# Autodesk Inventor assembly: 조립품2
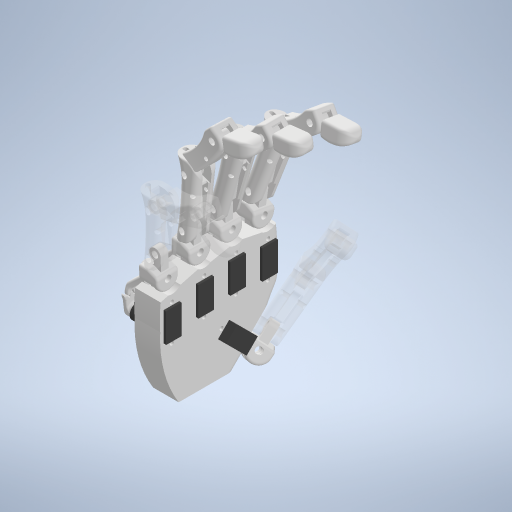
[picture p0: Inventor's stored thumbnail of the model, 512x512]
Saved by Autodesk Inventor 2024 (Build 280153000, 153)
## iProperties
Created: 2023-05-16
Part Number: 조립품2
Document SubType Name: Assembly
Designer: Lenovo
Author: Lenovo
## Documents named in this file (12)
- C:\Users\Lenovo\OneDrive\바탕 화면\로봇손\조립품2.iam
- C:\Users\Lenovo\OneDrive\바탕 화면\로봇손\손바닥.ipt
- C:\Users\Lenovo\OneDrive\바탕 화면\로봇손\손바닥 모터.ipt
- C:\Users\Lenovo\OneDrive\바탕 화면\로봇손\2,4 아래.ipt
- C:\Users\Lenovo\OneDrive\바탕 화면\로봇손\손바닥 위 -2.ipt
- C:\Users\Lenovo\OneDrive\바탕 화면\로봇손\3 아래.ipt
- C:\Users\Lenovo\OneDrive\바탕 화면\로봇손\중간.ipt
- C:\Users\Lenovo\OneDrive\바탕 화면\로봇손\위.ipt
- C:\Users\Lenovo\OneDrive\바탕 화면\로봇손\손바닥 위.ipt
- C:\Users\Lenovo\OneDrive\바탕 화면\로봇손\5 아래.ipt
- C:\Users\Lenovo\OneDrive\바탕 화면\로봇손\엄지 기어 -2.ipt
- C:\Users\Lenovo\OneDrive\바탕 화면\로봇손\손가락 기어.ipt
## Components (31 placed, 11 different names)
1. 손바닥:1 — 메이트:17, 메이트:18, 메이트:24, 메이트:27, 메이트:30, 메이트:36, 메이트:51, 메이트:52, 메이트:53, 메이트:54, 메이트:83, 메이트:84, 메이트:85, 메이트:86, 메이트:87, 메이트:88, 메이트:91, 메이트:92, 메이트:93, 메이트:96, 메이트:97, 메이트:98, 메이트:99, 메이트:100, 메이트:101
2. 손바닥 모터:4 — 메이트:17, 메이트:18, 메이트:36, 메이트:103, 메이트:107
3. 손바닥 모터:5 — 메이트:24, 메이트:27, 메이트:30, 메이트:102, 메이트:106
4. 손바닥 위 -2:4 — 메이트:79, 메이트:80, 메이트:83, 메이트:84
5. 중간:1 — 메이트:49, 메이트:50, 메이트:81, 메이트:82
6. 위:1 — 메이트:49, 메이트:50
7. 손바닥 위:1 — 메이트:51, 메이트:53, 메이트:57, 메이트:59
8. 손바닥 위:2 — 메이트:52, 메이트:54, 메이트:55, 메이트:56
9. 2,4 아래:2 — 메이트:57, 메이트:59, 메이트:65, 메이트:69
10. 2,4 아래:3 — 메이트:63, 메이트:67, 메이트:89
11. 5 아래:1 — 메이트:55, 메이트:56, 메이트:66, 메이트:70
12. 3 아래:2 — 메이트:64, 메이트:68, 메이트:90
13. 중간:2 — 메이트:63, 메이트:67, 메이트:71, 메이트:75
14. 중간:3 — 메이트:64, 메이트:68, 메이트:72, 메이트:76
15. 중간:4 — 메이트:65, 메이트:69, 메이트:73, 메이트:77
16. 중간:5 — 메이트:66, 메이트:70, 메이트:74, 메이트:78
17. 위:2 — 메이트:74, 메이트:78
18. 위:3 — 메이트:73, 메이트:77
19. 위:4 — 메이트:72, 메이트:76
20. 위:5 — 메이트:71, 메이트:75
21. 5 아래:2 — 메이트:79, 메이트:80, 메이트:81, 메이트:82
22. 손바닥 위:3 — 메이트:86, 메이트:87, 메이트:89
23. 손바닥 위:4 — 메이트:85, 메이트:88, 메이트:90
24. 손바닥 모터:9 — 메이트:91, 메이트:92, 메이트:93, 메이트:94, 메이트:95
25. 엄지 기어 -2:1 — 메이트:94, 메이트:95
26. 손바닥 모터:10 — 메이트:96, 메이트:97, 메이트:101, 메이트:104, 메이트:108
27. 손바닥 모터:11 — 메이트:98, 메이트:99, 메이트:100, 메이트:105, 메이트:109
28. 손가락 기어:1 — 메이트:102, 메이트:106
29. 손가락 기어:2 — 메이트:103, 메이트:107
30. 손가락 기어:3 — 메이트:104, 메이트:108
31. 손가락 기어:4 — 메이트:105, 메이트:109
## Relationships (63: Mate 63)
- 메이트:17 [Mate]: 손바닥:1 ↔ 손바닥 모터:4
- 메이트:18 [Mate]: 손바닥:1 ↔ 손바닥 모터:4
- 메이트:24 [Mate]: 손바닥:1 ↔ 손바닥 모터:5
- 메이트:27 [Mate]: 손바닥:1 ↔ 손바닥 모터:5
- 메이트:30 [Mate]: 손바닥:1 ↔ 손바닥 모터:5
- 메이트:36 [Mate]: 손바닥:1 ↔ 손바닥 모터:4
- 메이트:49 [Mate]: 중간:1 ↔ 위:1
- 메이트:50 [Mate] (0.5 mm): 중간:1 ↔ 위:1
- 메이트:51 [Mate]: 손바닥:1 ↔ 손바닥 위:1
- 메이트:52 [Mate]: 손바닥:1 ↔ 손바닥 위:2
- 메이트:53 [Mate] (0.5 mm): 손바닥:1 ↔ 손바닥 위:1
- 메이트:54 [Mate] (0.5 mm): 손바닥:1 ↔ 손바닥 위:2
- 메이트:55 [Mate]: 손바닥 위:2 ↔ 5 아래:1
- 메이트:56 [Mate] (0.5 mm): 손바닥 위:2 ↔ 5 아래:1
- 메이트:57 [Mate]: 손바닥 위:1 ↔ 2,4 아래:2
- 메이트:59 [Mate] (0.5 mm): 손바닥 위:1 ↔ 2,4 아래:2
- 메이트:63 [Mate]: 2,4 아래:3 ↔ 중간:2
- 메이트:64 [Mate]: 3 아래:2 ↔ 중간:3
- 메이트:65 [Mate]: 2,4 아래:2 ↔ 중간:4
- 메이트:66 [Mate]: 5 아래:1 ↔ 중간:5
- 메이트:67 [Mate] (0.5 mm): 2,4 아래:3 ↔ 중간:2
- 메이트:68 [Mate] (0.5 mm): 3 아래:2 ↔ 중간:3
- 메이트:69 [Mate] (0.5 mm): 2,4 아래:2 ↔ 중간:4
- 메이트:70 [Mate] (0.5 mm): 5 아래:1 ↔ 중간:5
- 메이트:71 [Mate]: 중간:2 ↔ 위:5
- 메이트:72 [Mate]: 중간:3 ↔ 위:4
- 메이트:73 [Mate]: 중간:4 ↔ 위:3
- 메이트:74 [Mate]: 중간:5 ↔ 위:2
- 메이트:75 [Mate] (0.5 mm): 중간:2 ↔ 위:5
- 메이트:76 [Mate] (0.5 mm): 중간:3 ↔ 위:4
- 메이트:77 [Mate] (0.5 mm): 중간:4 ↔ 위:3
- 메이트:78 [Mate] (0.5 mm): 중간:5 ↔ 위:2
- 메이트:79 [Mate]: 손바닥 위 -2:4 ↔ 5 아래:2
- 메이트:80 [Mate] (0.5 mm): 손바닥 위 -2:4 ↔ 5 아래:2
- 메이트:81 [Mate]: 중간:1 ↔ 5 아래:2
- 메이트:82 [Mate] (0.5 mm): 중간:1 ↔ 5 아래:2
- 메이트:83 [Mate]: 손바닥:1 ↔ 손바닥 위 -2:4
- 메이트:84 [Mate] (0.5 mm): 손바닥:1 ↔ 손바닥 위 -2:4
- 메이트:85 [Mate]: 손바닥:1 ↔ 손바닥 위:4
- 메이트:86 [Mate]: 손바닥:1 ↔ 손바닥 위:3
- 메이트:87 [Mate] (0.5 mm): 손바닥:1 ↔ 손바닥 위:3
- 메이트:88 [Mate] (0.5 mm): 손바닥:1 ↔ 손바닥 위:4
- 메이트:89 [Mate]: 2,4 아래:3 ↔ 손바닥 위:3
- 메이트:90 [Mate]: 3 아래:2 ↔ 손바닥 위:4
- 메이트:91 [Mate]: 손바닥:1 ↔ 손바닥 모터:9
- 메이트:92 [Mate]: 손바닥:1 ↔ 손바닥 모터:9
- 메이트:93 [Mate]: 손바닥:1 ↔ 손바닥 모터:9
- 메이트:94 [Mate]: 손바닥 모터:9 ↔ 엄지 기어 -2:1
- 메이트:95 [Mate] (0.5 mm): 손바닥 모터:9 ↔ 엄지 기어 -2:1
- 메이트:96 [Mate]: 손바닥:1 ↔ 손바닥 모터:10
- 메이트:97 [Mate]: 손바닥:1 ↔ 손바닥 모터:10
- 메이트:98 [Mate]: 손바닥:1 ↔ 손바닥 모터:11
- 메이트:99 [Mate]: 손바닥:1 ↔ 손바닥 모터:11
- 메이트:100 [Mate]: 손바닥:1 ↔ 손바닥 모터:11
- 메이트:101 [Mate]: 손바닥:1 ↔ 손바닥 모터:10
- 메이트:102 [Mate]: 손바닥 모터:5 ↔ 손가락 기어:1
- 메이트:103 [Mate]: 손바닥 모터:4 ↔ 손가락 기어:2
- 메이트:104 [Mate]: 손바닥 모터:10 ↔ 손가락 기어:3
- 메이트:105 [Mate]: 손바닥 모터:11 ↔ 손가락 기어:4
- 메이트:106 [Mate] (0.5 mm): 손바닥 모터:5 ↔ 손가락 기어:1
- 메이트:107 [Mate] (0.5 mm): 손바닥 모터:4 ↔ 손가락 기어:2
- 메이트:108 [Mate] (0.5 mm): 손바닥 모터:10 ↔ 손가락 기어:3
- 메이트:109 [Mate] (0.5 mm): 손바닥 모터:11 ↔ 손가락 기어:4
